# Autodesk Inventor assembly: matrix_V2
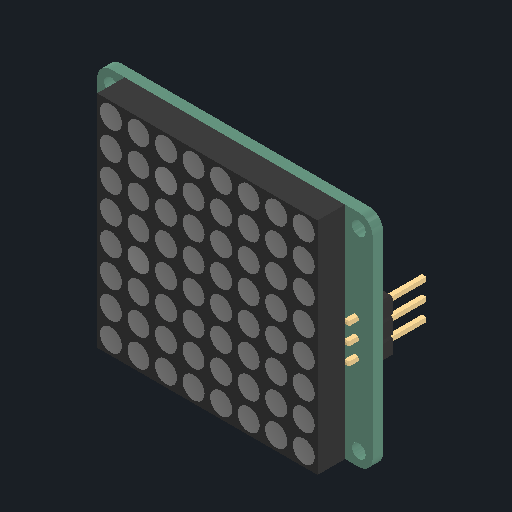
[picture p0: Inventor's stored thumbnail of the model, 512x512]
Saved by Autodesk Inventor 2026.1 (Build 301233000, 233)
## iProperties
Created: 2025-11-14
Part Number: matrix_V2
Document SubType Name: Assembly
Designer: micyg
Author: micyg
## Documents named in this file (3)
- C:\Users\micyg\Projects\virtual_pet\VirtualBlob\Mechanical\matrix\matrix_V2.iam
- C:\Users\micyg\Projects\virtual_pet\VirtualBlob\Mechanical\boards\MatrixBoard\MatrixBoard_0_0_0\MatrixBoard.iam
- C:\Users\micyg\Projects\virtual_pet\VirtualBlob\Mechanical\matrix\matrixDiffuser.ipt
## Components (2 placed, 2 different names)
1. MatrixBoard:1 [sub-assembly] — Zestawiające:1, Równoległe:1, Równoległe:2
2. matrixDiffuser:1 — Zestawiające:1, Równoległe:1, Równoległe:2
## Relationships (3: Flush 2, Mate 1)
- Zestawiające:1 [Mate]: MatrixBoard:1 ↔ matrixDiffuser:1
- Równoległe:1 [Flush]: MatrixBoard:1 ↔ matrixDiffuser:1
- Równoległe:2 [Flush] (4 mm): MatrixBoard:1 ↔ matrixDiffuser:1
